# Autodesk Inventor assembly: Assembly_Cube_Kinematic_Mirrormount_Thorlabs_90_PRO_magnetic_v3
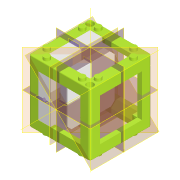
[picture p0: Inventor's stored thumbnail of the model, 180x180]
Saved by Autodesk Inventor 2022 (Build 260153000, 153)
## iProperties
Created: 2021-11-15
Part Number: Assembly_Cube_Kinematic_Mirrormount_Thorlabs_90_PRO_magnetic_v3
Document SubType Name: Assembly
Designer: diederichbenedict
Author: diederichbenedict
## Documents named in this file (5)
- C:\Users\diederichbenedict\Dropbox\Dokumente\Promotion\PROJECTS\openUC2-CAD\INVENTOR\Assembly_Cube_Kinematic_Mirrormount_Thorlabs_90_PRO_magnetic_v3.iam
- C:\Users\diederichbenedict\Dropbox\Dokumente\Promotion\PROJECTS\openUC2-CAD\INVENTOR\Assembly_Cube_empty_IM_v3.iam
- C:\Users\diederichbenedict\Dropbox\Dokumente\Promotion\PROJECTS\openUC2-CAD\INVENTOR\00_Thorlabs_PF10-03-P01-Step.ipt
- C:\Users\diederichbenedict\Dropbox\Dokumente\Promotion\PROJECTS\openUC2-CAD\INVENTOR\OLD\20_Cube_Insert_Kinematic_Mirror_90_pro_v3.ipt
- C:\Users\diederichbenedict\Dropbox\Dokumente\Promotion\PROJECTS\openUC2-CAD\INVENTOR\20_Cube_Insert_Kinematic_Thorlabs_1inch_pro_magnetic.ipt
## Components (4 placed, 4 different names)
1. Assembly_Cube_empty_IM_v3:1 [sub-assembly] — Mate:1, Mate:2, Mate:3, Mate:4, Angle:1, Angle:2, Mate:5
2. 00_Thorlabs_PF10-03-P01-Step:1 — Mate:1, Insert:1
3. 20_Cube_Insert_Kinematic_Mirror_90_pro_v3:1 — Mate:2, Mate:3, Mate:4, Angle:1, Angle:2, Mate:5, Flush:1, Flush:2
4. 20_Cube_Insert_Kinematic_Thorlabs_1inch_pro_magnetic:1 — Flush:1, Flush:2, Insert:1
## Relationships (10: Mate 5, Angle 2, Flush 2, Insert 1)
- Mate:1: Assembly_Cube_empty_IM_v3:1 ↔ 00_Thorlabs_PF10-03-P01-Step:1
- Mate:2: Assembly_Cube_empty_IM_v3:1 ↔ 20_Cube_Insert_Kinematic_Mirror_90_pro_v3:1
- Mate:3: Assembly_Cube_empty_IM_v3:1 ↔ 20_Cube_Insert_Kinematic_Mirror_90_pro_v3:1
- Mate:4: Assembly_Cube_empty_IM_v3:1 ↔ 20_Cube_Insert_Kinematic_Mirror_90_pro_v3:1
- Angle:1 (0 deg): Assembly_Cube_empty_IM_v3:1 ↔ 20_Cube_Insert_Kinematic_Mirror_90_pro_v3:1
- Angle:2 (0 deg): Assembly_Cube_empty_IM_v3:1 ↔ 20_Cube_Insert_Kinematic_Mirror_90_pro_v3:1
- Mate:5: Assembly_Cube_empty_IM_v3:1 ↔ 20_Cube_Insert_Kinematic_Mirror_90_pro_v3:1
- Flush:1: 20_Cube_Insert_Kinematic_Mirror_90_pro_v3:1 ↔ 20_Cube_Insert_Kinematic_Thorlabs_1inch_pro_magnetic:1
- Flush:2 (2 mm): 20_Cube_Insert_Kinematic_Mirror_90_pro_v3:1 ↔ 20_Cube_Insert_Kinematic_Thorlabs_1inch_pro_magnetic:1
- Insert:1: 00_Thorlabs_PF10-03-P01-Step:1 ↔ 20_Cube_Insert_Kinematic_Thorlabs_1inch_pro_magnetic:1
